# Autodesk Inventor assembly: center_2p_female
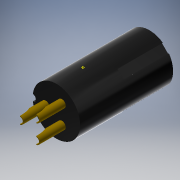
[picture p0: Inventor's stored thumbnail of the model, 180x180]
Saved by Autodesk Inventor 2018 (Build 220112000, 112)
## iProperties
Created: 2019-04-17
Part Number: center_2p_female
Document SubType Name: Assembly
Designer: ZEUSLAP
Author: ZEUSLAP
## Documents named in this file (3)
- C:\Users\Vadim\Desktop\sp16-waterproof-connector-1.snapshot.3\parts\center_3p_female.iam
- C:\Users\Vadim\Desktop\sp16-waterproof-connector-1.snapshot.3\parts\pin_1.8mm.ipt
- C:\Users\Vadim\Desktop\sp16-waterproof-connector-1.snapshot.3\parts\center_3p_female_body.ipt
## Components (4 placed, 2 different names)
1. center_2p_female_body:1 — Angle:1, Angle:2, Angle:3, Mate:2, Angle:4, Flush:2, Mate:3, Angle:7, Mate:4, Angle:8
2. pin_1.8mm:1 — Angle:3, Mate:2, Flush:1, Angle:5, Flush:2, Flush:3
3. pin_1.8mm:2 — Angle:2, Flush:1, Angle:6, Mate:3
4. pin_1.8mm:3 — Angle:7, Mate:4, Angle:8, Flush:3
## Relationships (14: Angle 8, Mate 3, Flush 3)
- Angle:1 (0 deg): center_2p_female_body:1
- Angle:2 (0 deg): center_2p_female_body:1 ↔ pin_1.8mm:2
- Angle:3 (0 deg): center_2p_female_body:1 ↔ pin_1.8mm:1
- Mate:2: center_2p_female_body:1 ↔ pin_1.8mm:1
- Flush:1: pin_1.8mm:1 ↔ pin_1.8mm:2
- Angle:4 (180 deg): center_2p_female_body:1
- Angle:5 (90 deg): pin_1.8mm:1
- Angle:6 (90 deg): pin_1.8mm:2
- Flush:2 (6 mm): center_2p_female_body:1 ↔ pin_1.8mm:1
- Mate:3: center_2p_female_body:1 ↔ pin_1.8mm:2
- Angle:7 (0 deg): center_2p_female_body:1 ↔ pin_1.8mm:3
- Mate:4: center_2p_female_body:1 ↔ pin_1.8mm:3
- Angle:8 (90 deg): center_2p_female_body:1 ↔ pin_1.8mm:3
- Flush:3: pin_1.8mm:1 ↔ pin_1.8mm:3
